# Autodesk Inventor assembly: Zassembly
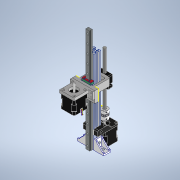
[picture p0: Inventor's stored thumbnail of the model, 180x180]
Saved by Autodesk Inventor 2022 (Build 260153000, 153)
## iProperties
Created: 2022-02-16
Part Number: Zassembly
Document SubType Name: Assembly
Designer: JK
Author: JK
## Documents named in this file (14)
- C:\Users\JK\Documents\Inventor\ScaraNema\Zassembly.iam
- C:\Users\JK\Documents\Inventor\ScaraNema\V-Slot 20x20.ipt
- C:\Users\JK\Documents\Inventor\ScaraNema\ACMEThread.ipt
- C:\Users\JK\Documents\Inventor\ScaraNema\Tr8NutDelrinplate.ipt
- C:\Users\JK\Documents\Inventor\ScaraNema\MOTOR_LONG.ipt
- C:\Users\JK\Documents\Inventor\ScaraNema\Flexible_Shaft_Coupling_5_to_8mm v7.iam
- C:\Users\JK\Documents\Inventor\ScaraNema\V-Slot 20x20\V-Slot 20x20-250.ipt
- C:\Users\JK\Documents\Inventor\ScaraNema\ConjuntoUnion90GradosPerfil2020.iam
- C:\Users\JK\Documents\Inventor\ScaraNema\Linear rail.ipt
- C:\Users\JK\Documents\Inventor\ScaraNema\MGN12H.ipt
- C:\Users\JK\Documents\Inventor\ScaraNema\Zcarriage.ipt
- C:\Users\JK\Documents\Inventor\ScaraNema\Zmotorsupport.ipt
- C:\Users\JK\Documents\Inventor\ScaraNema\elbowmotorsupport.ipt
- C:\Users\JK\Documents\Inventor\ScaraNema\MOTOR.ipt
## Components (13 placed, 12 different names)
1. V-Slot 20x20-250:1 — Nivelación:1, Coincidencia:1, Nivelación:2, Nivelación:4, Coincidencia:9, Nivelación:5, Coincidencia:10, Nivelación:7, Coincidencia:11, Nivelación:8, Nivelación:10
2. Wał:1 — Coincidencia:2, Coincidencia:3, Coincidencia:8
3. Tr8NutDelrinplate:1 — Coincidencia:3, Ángulo:2, Coincidencia:14, Coincidencia:15, Coincidencia:16
4. MOTOR_LONG:1 — Nivelación:1, Coincidencia:1, Nivelación:2, Coincidencia:2, Coincidencia:7, Nivelación:3, Coincidencia:18, Coincidencia:19, Ángulo:3
5. Flexible_Shaft_Coupling_5_to_8mm v7:1 [sub-assembly] — Coincidencia:7, Nivelación:3, Coincidencia:8
6. ConjuntoUnion90GradosPerfil2020:1 [sub-assembly] — Nivelación:6, Coincidencia:10, Nivelación:7
7. ConjuntoUnion90GradosPerfil2020:2 [sub-assembly] — Nivelación:4, Coincidencia:9, Nivelación:5, Nivelación:6
8. Linear rail:1 — Coincidencia:11, Nivelación:8, Ángulo:1, Nivelación:9, Coincidencia:12, Nivelación:10, Ángulo:2, Ángulo:4
9. MGN12H:1 — Ángulo:1, Nivelación:9, Coincidencia:12, Coincidencia:13, Coincidencia:17
10. Zcarriage:1 — Coincidencia:13, Coincidencia:14, Coincidencia:15, Coincidencia:16, Coincidencia:17, Coincidencia:20, Coincidencia:21, Coincidencia:22
11. Zmotorsupport:1 — Coincidencia:18, Coincidencia:19, Ángulo:3
12. elbowmotorsupport:1 — Coincidencia:20, Coincidencia:21, Coincidencia:22, Coincidencia:23, Coincidencia:24
13. MOTOR:1 — Coincidencia:23, Coincidencia:24, Ángulo:4
## Relationships (35: Mate 21, Flush 10, Angle 4)
- Nivelación:1 [Flush]: V-Slot 20x20-250:1 ↔ MOTOR_LONG:1
- Coincidencia:1 [Mate]: V-Slot 20x20-250:1 ↔ MOTOR_LONG:1
- Nivelación:2 [Flush] (-10.75 mm): V-Slot 20x20-250:1 ↔ MOTOR_LONG:1
- Coincidencia:2 [Mate]: Wał:1 ↔ MOTOR_LONG:1
- Coincidencia:3 [Mate]: Wał:1 ↔ Tr8NutDelrinplate:1
- Coincidencia:7 [Mate]: MOTOR_LONG:1 ↔ Flexible_Shaft_Coupling_5_to_8mm v7:1
- Nivelación:3 [Flush]: MOTOR_LONG:1 ↔ Flexible_Shaft_Coupling_5_to_8mm v7:1
- Coincidencia:8 [Mate]: Wał:1 ↔ Flexible_Shaft_Coupling_5_to_8mm v7:1
- Nivelación:4 [Flush]: V-Slot 20x20-250:1 ↔ ConjuntoUnion90GradosPerfil2020:2
- Coincidencia:9 [Mate]: V-Slot 20x20-250:1 ↔ ConjuntoUnion90GradosPerfil2020:2
- Nivelación:5 [Flush]: V-Slot 20x20-250:1 ↔ ConjuntoUnion90GradosPerfil2020:2
- Nivelación:6 [Flush]: ConjuntoUnion90GradosPerfil2020:1 ↔ ConjuntoUnion90GradosPerfil2020:2
- Coincidencia:10 [Mate]: V-Slot 20x20-250:1 ↔ ConjuntoUnion90GradosPerfil2020:1
- Nivelación:7 [Flush]: V-Slot 20x20-250:1 ↔ ConjuntoUnion90GradosPerfil2020:1
- Coincidencia:11 [Mate]: V-Slot 20x20-250:1 ↔ Linear rail:1
- Nivelación:8 [Flush] (4 mm): V-Slot 20x20-250:1 ↔ Linear rail:1
- Ángulo:1 [Angle] (180 deg): Linear rail:1 ↔ MGN12H:1
- Nivelación:9 [Flush] (-7.5 mm): Linear rail:1 ↔ MGN12H:1
- Coincidencia:12 [Mate]: Linear rail:1 ↔ MGN12H:1
- Nivelación:10 [Flush]: V-Slot 20x20-250:1 ↔ Linear rail:1
- Coincidencia:13 [Mate]: MGN12H:1 ↔ Zcarriage:1
- Ángulo:2 [Angle] (0 deg): Tr8NutDelrinplate:1 ↔ Linear rail:1
- Coincidencia:14 [Mate]: Tr8NutDelrinplate:1 ↔ Zcarriage:1
- Coincidencia:15 [Mate]: Tr8NutDelrinplate:1 ↔ Zcarriage:1
- Coincidencia:16 [Mate]: Tr8NutDelrinplate:1 ↔ Zcarriage:1
- Coincidencia:17 [Mate]: MGN12H:1 ↔ Zcarriage:1
- Coincidencia:18 [Mate]: MOTOR_LONG:1 ↔ Zmotorsupport:1
- Coincidencia:19 [Mate]: MOTOR_LONG:1 ↔ Zmotorsupport:1
- Ángulo:3 [Angle] (0 deg): MOTOR_LONG:1 ↔ Zmotorsupport:1
- Coincidencia:20 [Mate]: Zcarriage:1 ↔ elbowmotorsupport:1
- Coincidencia:21 [Mate]: Zcarriage:1 ↔ elbowmotorsupport:1
- Coincidencia:22 [Mate]: Zcarriage:1 ↔ elbowmotorsupport:1
- Coincidencia:23 [Mate]: elbowmotorsupport:1 ↔ MOTOR:1
- Coincidencia:24 [Mate]: elbowmotorsupport:1 ↔ MOTOR:1
- Ángulo:4 [Angle] (0 deg): Linear rail:1 ↔ MOTOR:1
